# Autodesk Inventor assembly: assembly
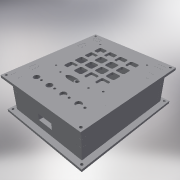
[picture p0: Inventor's stored thumbnail of the model, 180x180]
Saved by Autodesk Inventor 2017 (Build 210142000, 142)
## iProperties
Created: 2017-05-22
Part Number: assembly
Document SubType Name: Assembly
Designer: Dominic Gaiero
Author: Dominic Gaiero
## Documents named in this file (8)
- C:\Users\Dominic Gaiero\Documents\projects\Arduino-MIDI-Controller\Inventor Files\MIDI_proj\assembly.iam
- C:\Users\Dominic Gaiero\Documents\projects\Arduino-MIDI-Controller\Inventor Files\MIDI_proj\boxBack.ipt
- C:\Users\Dominic Gaiero\Documents\projects\Arduino-MIDI-Controller\Inventor Files\MIDI_proj\boxBottom.ipt
- C:\Users\Dominic Gaiero\Documents\projects\Arduino-MIDI-Controller\Inventor Files\MIDI_proj\boxFront.ipt
- C:\Users\Dominic Gaiero\Documents\projects\Arduino-MIDI-Controller\Inventor Files\MIDI_proj\boxSide.ipt
- C:\Users\Dominic Gaiero\Documents\projects\Arduino-MIDI-Controller\Inventor Files\MIDI_proj\boxTop.ipt
- C:\Users\Dominic Gaiero\Documents\projects\Arduino-MIDI-Controller\Inventor Files\MIDI_proj\trellisCaptiveBottom.ipt
- C:\Users\Dominic Gaiero\Documents\projects\Arduino-MIDI-Controller\Inventor Files\MIDI_proj\trellisCaptiveTop.ipt
## Components (8 placed, 7 different names)
1. boxBack:1 — Mate:4, Mate:5, Mate:6, Flush:2, Mate:10, Flush:4
2. boxBottom:1 — Mate:1, Mate:2, Mate:3, Mate:4, Mate:5, Mate:6
3. boxFront:1 — Mate:1, Mate:2, Mate:3, Flush:3, Flush:5, Flush:6, Mate:18
4. boxTop:1 — Mate:11, Mate:12, Mate:13, Mate:16, Mate:17, Mate:18
5. boxSide:1 — Mate:10, Flush:5, Flush:6
6. boxSide:2 — Flush:2, Flush:3, Flush:4, Mate:16, Mate:17
7. trellisCaptiveBottom:1 — Mate:11, Mate:12, Mate:13, Mate:14, Mate:15, Flush:7
8. trellisCaptiveTop:1 — Mate:14, Mate:15, Flush:7
## Relationships (21: Mate 15, Flush 6)
- Mate:1: boxBottom:1 ↔ boxFront:1
- Mate:2: boxBottom:1 ↔ boxFront:1
- Mate:3: boxBottom:1 ↔ boxFront:1
- Mate:4: boxBack:1 ↔ boxBottom:1
- Mate:5: boxBack:1 ↔ boxBottom:1
- Mate:6: boxBack:1 ↔ boxBottom:1
- Flush:2: boxBack:1 ↔ boxSide:2
- Mate:10: boxBack:1 ↔ boxSide:1
- Flush:3: boxFront:1 ↔ boxSide:2
- Flush:4: boxBack:1 ↔ boxSide:2
- Flush:5: boxFront:1 ↔ boxSide:1
- Flush:6: boxFront:1 ↔ boxSide:1
- Mate:11: boxTop:1 ↔ trellisCaptiveBottom:1
- Mate:12: boxTop:1 ↔ trellisCaptiveBottom:1
- Mate:13: boxTop:1 ↔ trellisCaptiveBottom:1
- Mate:14: trellisCaptiveBottom:1 ↔ trellisCaptiveTop:1
- Mate:15: trellisCaptiveBottom:1 ↔ trellisCaptiveTop:1
- Flush:7: trellisCaptiveBottom:1 ↔ trellisCaptiveTop:1
- Mate:16: boxTop:1 ↔ boxSide:2
- Mate:17: boxTop:1 ↔ boxSide:2
- Mate:18: boxFront:1 ↔ boxTop:1
